# Autodesk Inventor assembly: PrintCameraPi
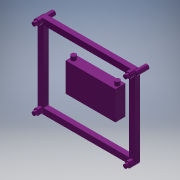
[picture p0: Inventor's stored thumbnail of the model, 180x180]
Saved by Autodesk Inventor 2018 (Build 220112000, 112)
## iProperties
Created: 2018-01-13
Part Number: PrintCameraPi
Document SubType Name: Assembly
Designer: Kyle-HP
Author: Kyle-HP
## Documents named in this file (3)
- C:\Users\Kyle-HP\Documents\Hackathon-2018\Inventor\Robot\PrintCameraPi.iam
- C:\Users\Kyle-HP\Documents\Hackathon-2018\Inventor\Robot\CameraMount.ipt
- C:\Users\Kyle-HP\Documents\Hackathon-2018\Inventor\Robot\PiMount.ipt
## Components (2 placed, 2 different names)
1. CameraMount:1 — Flush:1
2. PiMount:1 — Flush:1
## Relationships (1: Flush 1)
- Flush:1: CameraMount:1 ↔ PiMount:1
